# Autodesk Inventor assembly: LuggageSubassembly
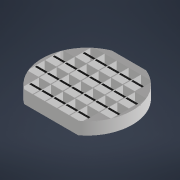
[picture p0: Inventor's stored thumbnail of the model, 180x180]
Saved by Autodesk Inventor 2021 (Build 250183000, 183)
## iProperties
Created: 2021-01-31
Part Number: LuggageSubassembly
Document SubType Name: Assembly
Designer: argon
Author: argon
## Documents named in this file (4)
- C:\Users\argon\OneDrive\Documents\GrabCAD\EngOne Maroons\Luggage Subassembly\LuggageSubassembly.iam
- C:\Users\argon\OneDrive\Documents\GrabCAD\EngOne Maroons\Luggage Subassembly\LuggageHoneyComb.ipt
- C:\Users\argon\OneDrive\Documents\GrabCAD\EngOne Maroons\Luggage Subassembly\LuggageStrapLong.ipt
- C:\Users\argon\OneDrive\Documents\GrabCAD\EngOne Maroons\Luggage Subassembly\LuggageStrapShort.ipt
## Components (5 placed, 3 different names)
1. LuggageHoneyComb:1 — Mate:1, Mate:2, Mate:3, Mate:4, Mate:5, Mate:6, Mate:7, Mate:8, Mate:9, Mate:10
2. LuggageStrapLong:1 — Flush:1, Flush:3, Mate:6, Mate:7, Mate:8
3. LuggageStrapShort:1 — Flush:2, Mate:9, Mate:10
4. LuggageStrapLong:2 — Flush:1, Mate:4, Mate:5
5. LuggageStrapShort:2 — Flush:2, Flush:3, Mate:1, Mate:2, Mate:3
## Relationships (13: Mate 10, Flush 3)
- Flush:1: LuggageStrapLong:1 ↔ LuggageStrapLong:2
- Flush:2: LuggageStrapShort:1 ↔ LuggageStrapShort:2
- Flush:3: LuggageStrapLong:1 ↔ LuggageStrapShort:2
- Mate:1: LuggageHoneyComb:1 ↔ LuggageStrapShort:2
- Mate:2: LuggageHoneyComb:1 ↔ LuggageStrapShort:2
- Mate:3: LuggageHoneyComb:1 ↔ LuggageStrapShort:2
- Mate:4: LuggageHoneyComb:1 ↔ LuggageStrapLong:2
- Mate:5: LuggageHoneyComb:1 ↔ LuggageStrapLong:2
- Mate:6: LuggageHoneyComb:1 ↔ LuggageStrapLong:1
- Mate:7: LuggageHoneyComb:1 ↔ LuggageStrapLong:1
- Mate:8: LuggageHoneyComb:1 ↔ LuggageStrapLong:1
- Mate:9: LuggageHoneyComb:1 ↔ LuggageStrapShort:1
- Mate:10: LuggageHoneyComb:1 ↔ LuggageStrapShort:1
